# Autodesk Inventor assembly: servo_frame_with_nuts
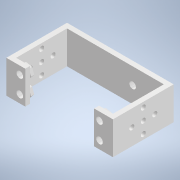
[picture p0: Inventor's stored thumbnail of the model, 180x180]
Saved by Autodesk Inventor 2021.4 (Build 254397000, 397)
## iProperties
Created: 2022-07-24
Part Number: servo_frame_with_nuts
Document SubType Name: Assembly
Designer: isamu
Author: isamu
## Documents named in this file (3)
- D:\personal_projects\robot\inventor\2021_export_exp\servo_frame_with_nuts.iam
- D:\personal_projects\robot\exports\frames\servo frame.ipt
- D:\personal_projects\robot\exports\screws\m4 nuts.ipt
## Components (5 placed, 2 different names)
1. servo frame:1 — Insert:1, Insert:2, Insert:3, Insert:4
2. m4 nuts:1 — Insert:1
3. m4 nuts:2 — Insert:3
4. m4 nuts:3 — Insert:4
5. m4 nuts:4 — Insert:2
## Relationships (4: Insert 4)
- Insert:1: servo frame:1 ↔ m4 nuts:1
- Insert:2: servo frame:1 ↔ m4 nuts:4
- Insert:3: servo frame:1 ↔ m4 nuts:2
- Insert:4: servo frame:1 ↔ m4 nuts:3
